# Autodesk Inventor assembly: AssemblyTest
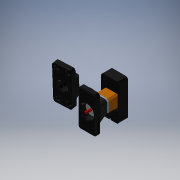
[picture p0: Inventor's stored thumbnail of the model, 180x180]
Saved by Autodesk Inventor 2019 (Build 230136000, 136)
## iProperties
Created: 2019-05-15
Part Number: AssemblyTest
Document SubType Name: Assembly
Designer: Iván
Author: Iván
## Documents named in this file (5)
- C:\Users\Ivan\Documents\GitHub\RMTestMachine\3DModel\AssemblyTest.iam
- C:\Users\Ivan\Documents\GitHub\RMTestMachine\3DModel\Imported Components\pieza1_correccion\pieza1_correccion.ipt
- C:\Users\Ivan\Documents\GitHub\RMTestMachine\3DModel\Imported Components\pieza2_correccion\pieza2_correccion.ipt
- C:\Users\Ivan\Documents\GitHub\RMTestMachine\3DModel\Imported Components\pieza3\pieza3.ipt
- C:\Users\Ivan\Documents\GitHub\RMTestMachine\3DModel\motor con reductora - escalado.ipt
## Components (4 placed, 4 different names)
1. pieza1_correccion:1
2. pieza2_correccion:1 — Mate:6, Angle:1, Mate:7
3. pieza3:1 — Mate:1, Mate:2, Mate:3, Mate:4, Mate:5, Angle:1
4. motor con reductora - escalado:1 — Mate:1, Mate:4, Mate:5, Mate:6, Mate:7
## Relationships (8: Mate 7, Angle 1)
- Mate:1: pieza3:1 ↔ motor con reductora - escalado:1
- Mate:2: pieza3:1
- Mate:3: pieza3:1
- Mate:4: pieza3:1 ↔ motor con reductora - escalado:1
- Mate:5: pieza3:1 ↔ motor con reductora - escalado:1
- Mate:6: pieza2_correccion:1 ↔ motor con reductora - escalado:1
- Angle:1 (0 deg): pieza2_correccion:1 ↔ pieza3:1
- Mate:7: pieza2_correccion:1 ↔ motor con reductora - escalado:1
